# Autodesk Inventor assembly: 二輪足回り
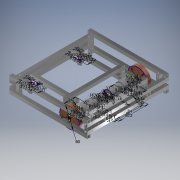
[picture p0: Inventor's stored thumbnail of the model, 180x180]
Saved by Autodesk Inventor 2018.2 (Build 222227000, 227)
## iProperties
Created: 2019-04-22
Part Number: 二輪足回り
Material: 一般
Document SubType Name: Assembly
Designer: Eiji Nishizawa
Author: Eiji Nishizawa
## Documents named in this file (14)
- D:\西澤　英志\OneDrive\CAD\二輪足回り\二輪足回り.iam
- D:\西澤　英志\OneDrive\CAD\二輪足回り\モーター100：1.iam
- D:\西澤　英志\OneDrive\CAD\二輪足回り\モーターパーツ１.ipt
- D:\西澤　英志\OneDrive\CAD\二輪足回り\モーターパーツ３.ipt
- D:\西澤　英志\OneDrive\CAD\二輪足回り\モーターパーツ２.ipt
- D:\西澤　英志\OneDrive\CAD\二輪足回り\スリットカラー.ipt
- D:\西澤　英志\OneDrive\CAD\二輪足回り\タイヤ.ipt
- D:\西澤　英志\OneDrive\CAD\二輪足回り\flontparts1.ipt
- D:\西澤　英志\OneDrive\CAD\二輪足回り\backparts1.ipt
- D:\西澤　英志\OneDrive\CAD\二輪足回り\f&bparts.ipt
- D:\西澤　英志\OneDrive\CAD\二輪足回り\sideparts.ipt
- D:\西澤　英志\OneDrive\CAD\二輪足回り\キャスター.ipt
- D:\西澤　英志\OneDrive\CAD\二輪足回り\角パーツ.ipt
- D:\西澤　英志\OneDrive\CAD\2018高専ロボコン\光センサー\光センサーケース.iam
## Components (33 placed, 13 different names)
1. モーター100：1:1 [sub-assembly] — 挿入:9, 挿入:10, 挿入:11, 挿入:12, 挿入:13, 挿入:14, 挿入:39
2. モーター100：1:2 [sub-assembly] — メイト:1, メイト:2, メイト:3, メイト:4, 挿入:27
3. モーターパーツ１:1 — 挿入:9, 挿入:10, 挿入:11, 挿入:12, 挿入:13, 挿入:14, 挿入:15, 挿入:16, 挿入:17, 挿入:18, 挿入:49, 挿入:50
4. モーターパーツ１:2 — メイト:1, メイト:2, メイト:3, メイト:4, 挿入:1, 挿入:2, 挿入:3, 挿入:4, 挿入:48, 挿入:51
5. モーターパーツ２:1 — 挿入:15, 挿入:16, 挿入:35
6. モーターパーツ２:2 — 挿入:17, 挿入:18, 挿入:31, 挿入:53
7. モーターパーツ２:3 — 挿入:3, 挿入:4, 挿入:32, 挿入:52
8. モーターパーツ２:4 — 挿入:1, 挿入:2, 挿入:36
9. スリットカラー:1 — 挿入:25, 挿入:26, 挿入:27
10. スリットカラー:2 — 挿入:37, 挿入:38, 挿入:39
11. タイヤ:1 — 挿入:25, 挿入:26
12. タイヤ:2 — 挿入:37, 挿入:38
13. flontparts1:1 — 挿入:32, 挿入:43, 挿入:54
14. flontparts1:2 — 挿入:31, 挿入:40, 挿入:55
15. backparts1:1 — 挿入:36, 挿入:42
16. backparts1:2 — 挿入:35, 挿入:41
17. f&bparts:1 — 挿入:41, 挿入:42, 挿入:46, 挿入:47, 挿入:56, 挿入:57, 挿入:58, 挿入:59, 挿入:64, 挿入:65
18. f&bparts:2 — 挿入:40, 挿入:43, 挿入:44, 挿入:45, 挿入:66, 挿入:67
19. sideparts:1 — 挿入:45, 挿入:46, 挿入:61, 挿入:62
20. sideparts:2 — 挿入:44, 挿入:47, 挿入:60, 挿入:63
21. モーターパーツ３:1 — 挿入:50, 挿入:51, 挿入:52, 挿入:53, 挿入:54, 挿入:55
22. モーターパーツ３:2 — 挿入:48, 挿入:49
23. キャスター:1 — 挿入:57, 挿入:58
24. キャスター:2 — 挿入:56, 挿入:59
25. 角パーツ:1 — 挿入:60, 挿入:67, 挿入:69, 挿入:74
26. 角パーツ:2 — 挿入:61, 挿入:66, 挿入:68, 挿入:75
27. 角パーツ:3 — 挿入:62, 挿入:65, 挿入:71, 挿入:76
28. 角パーツ:4 — 挿入:63, 挿入:64, 挿入:70, 挿入:77
29. f&bparts:3 — 挿入:70, 挿入:71, 挿入:78, 挿入:79
30. f&bparts:4 — 挿入:68, 挿入:69, 挿入:72, 挿入:73
31. sideparts:3 — 挿入:72, 挿入:75, 挿入:76, 挿入:79
32. sideparts:4 — 挿入:73, 挿入:74, 挿入:77, 挿入:78
33. 光センサーケース:1 [sub-assembly]
## Relationships (68: Insert 64, Mate 4)
- メイト:1 [Mate]: モーター100：1:2 ↔ モーターパーツ１:2
- メイト:2 [Mate]: モーター100：1:2 ↔ モーターパーツ１:2
- メイト:3 [Mate]: モーター100：1:2 ↔ モーターパーツ１:2
- メイト:4 [Mate]: モーター100：1:2 ↔ モーターパーツ１:2
- 挿入:1 [Insert]: モーターパーツ１:2 ↔ モーターパーツ２:4
- 挿入:2 [Insert]: モーターパーツ１:2 ↔ モーターパーツ２:4
- 挿入:3 [Insert]: モーターパーツ１:2 ↔ モーターパーツ２:3
- 挿入:4 [Insert]: モーターパーツ１:2 ↔ モーターパーツ２:3
- 挿入:9 [Insert]: モーター100：1:1 ↔ モーターパーツ１:1
- 挿入:10 [Insert]: モーター100：1:1 ↔ モーターパーツ１:1
- 挿入:11 [Insert]: モーター100：1:1 ↔ モーターパーツ１:1
- 挿入:12 [Insert]: モーター100：1:1 ↔ モーターパーツ１:1
- 挿入:13 [Insert]: モーター100：1:1 ↔ モーターパーツ１:1
- 挿入:14 [Insert]: モーター100：1:1 ↔ モーターパーツ１:1
- 挿入:15 [Insert]: モーターパーツ１:1 ↔ モーターパーツ２:1
- 挿入:16 [Insert]: モーターパーツ１:1 ↔ モーターパーツ２:1
- 挿入:17 [Insert]: モーターパーツ１:1 ↔ モーターパーツ２:2
- 挿入:18 [Insert]: モーターパーツ１:1 ↔ モーターパーツ２:2
- 挿入:25 [Insert]: スリットカラー:1 ↔ タイヤ:1
- 挿入:26 [Insert]: スリットカラー:1 ↔ タイヤ:1
- 挿入:27 [Insert]: モーター100：1:2 ↔ スリットカラー:1
- 挿入:31 [Insert]: モーターパーツ２:2 ↔ flontparts1:2
- 挿入:32 [Insert]: モーターパーツ２:3 ↔ flontparts1:1
- 挿入:35 [Insert]: モーターパーツ２:1 ↔ backparts1:2
- 挿入:36 [Insert]: モーターパーツ２:4 ↔ backparts1:1
- 挿入:37 [Insert]: スリットカラー:2 ↔ タイヤ:2
- 挿入:38 [Insert]: スリットカラー:2 ↔ タイヤ:2
- 挿入:39 [Insert]: モーター100：1:1 ↔ スリットカラー:2
- 挿入:40 [Insert]: flontparts1:2 ↔ f&bparts:2
- 挿入:41 [Insert]: backparts1:2 ↔ f&bparts:1
- 挿入:42 [Insert]: backparts1:1 ↔ f&bparts:1
- 挿入:43 [Insert]: flontparts1:1 ↔ f&bparts:2
- 挿入:44 [Insert]: f&bparts:2 ↔ sideparts:2
- 挿入:45 [Insert]: f&bparts:2 ↔ sideparts:1
- 挿入:46 [Insert]: f&bparts:1 ↔ sideparts:1
- 挿入:47 [Insert]: f&bparts:1 ↔ sideparts:2
- 挿入:48 [Insert]: モーターパーツ１:2 ↔ モーターパーツ３:2
- 挿入:49 [Insert]: モーターパーツ１:1 ↔ モーターパーツ３:2
- 挿入:50 [Insert]: モーターパーツ１:1 ↔ モーターパーツ３:1
- 挿入:51 [Insert]: モーターパーツ１:2 ↔ モーターパーツ３:1
- 挿入:52 [Insert]: モーターパーツ２:3 ↔ モーターパーツ３:1
- 挿入:53 [Insert]: モーターパーツ２:2 ↔ モーターパーツ３:1
- 挿入:54 [Insert]: flontparts1:1 ↔ モーターパーツ３:1
- 挿入:55 [Insert]: flontparts1:2 ↔ モーターパーツ３:1
- 挿入:56 [Insert]: f&bparts:1 ↔ キャスター:2
- 挿入:57 [Insert]: f&bparts:1 ↔ キャスター:1
- 挿入:58 [Insert]: f&bparts:1 ↔ キャスター:1
- 挿入:59 [Insert]: f&bparts:1 ↔ キャスター:2
- 挿入:60 [Insert]: sideparts:2 ↔ 角パーツ:1
- 挿入:61 [Insert]: sideparts:1 ↔ 角パーツ:2
- 挿入:62 [Insert]: sideparts:1 ↔ 角パーツ:3
- 挿入:63 [Insert]: sideparts:2 ↔ 角パーツ:4
- 挿入:64 [Insert]: f&bparts:1 ↔ 角パーツ:4
- 挿入:65 [Insert]: f&bparts:1 ↔ 角パーツ:3
- 挿入:66 [Insert]: f&bparts:2 ↔ 角パーツ:2
- 挿入:67 [Insert]: f&bparts:2 ↔ 角パーツ:1
- 挿入:68 [Insert]: 角パーツ:2 ↔ f&bparts:4
- 挿入:69 [Insert]: 角パーツ:1 ↔ f&bparts:4
- 挿入:70 [Insert]: 角パーツ:4 ↔ f&bparts:3
- 挿入:71 [Insert]: 角パーツ:3 ↔ f&bparts:3
- 挿入:72 [Insert]: f&bparts:4 ↔ sideparts:3
- 挿入:73 [Insert]: f&bparts:4 ↔ sideparts:4
- 挿入:74 [Insert]: 角パーツ:1 ↔ sideparts:4
- 挿入:75 [Insert]: 角パーツ:2 ↔ sideparts:3
- 挿入:76 [Insert]: 角パーツ:3 ↔ sideparts:3
- 挿入:77 [Insert]: 角パーツ:4 ↔ sideparts:4
- 挿入:78 [Insert]: f&bparts:3 ↔ sideparts:4
- 挿入:79 [Insert]: f&bparts:3 ↔ sideparts:3
